# Autodesk Inventor assembly: Cross Shaft
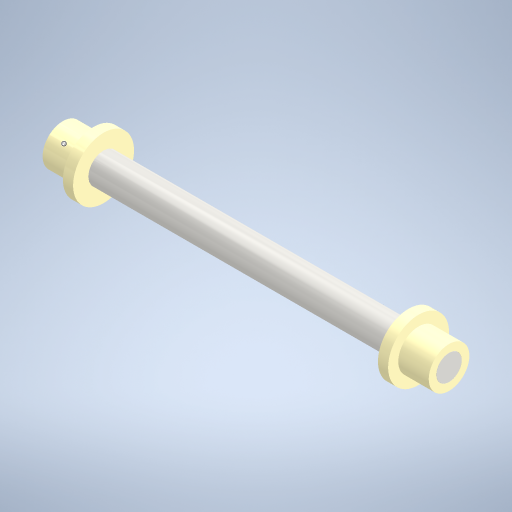
[picture p0: Inventor's stored thumbnail of the model, 512x512]
Saved by Autodesk Inventor 2024 (Build 280153000, 153)
## iProperties
Created: 2023-11-21
Part Number: Cross Shaft
Document SubType Name: Assembly
Designer: Greg
Author: Greg
## Documents named in this file (3)
- C:\Users\greg\Documents\Inventor\Capstone\Chalk Applicator\Cross Shaft.iam
- C:\Users\greg\Documents\Inventor\Capstone\Chalk Applicator\Shaft1.ipt
- C:\Users\greg\Documents\Inventor\Capstone\Chalk Applicator\Nylon Slider.ipt
## Components (3 placed, 2 different names)
1. Shaft:1 — Insert:1, Insert:2
2. Nylon Slider:1 — Insert:1
3. Nylon Slider:2 — Insert:2
## Relationships (2: Insert 2)
- Insert:1: Shaft:1 ↔ Nylon Slider:1
- Insert:2: Shaft:1 ↔ Nylon Slider:2
